# Autodesk Inventor assembly: P3_device(Main)
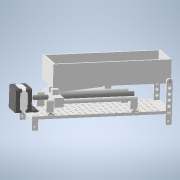
[picture p0: Inventor's stored thumbnail of the model, 180x180]
Saved by Autodesk Inventor 2021 (Build 250183000, 183)
## iProperties
Created: 2021-02-05
Part Number: P3_device(Main)
Document SubType Name: Assembly
Designer: chris
Author: chris
## Documents named in this file (13)
- C:\Users\chris\Desktop\Mon-38_P3_CAD_Files\Project 3 Device\P3_device(Main).iam
- C:\Users\chris\Desktop\Mon-38_P3_CAD_Files\Project 3 Device\Q-Bot baseplate\Mounting Platform.iam
- C:\Users\chris\Desktop\Mon-38_P3_CAD_Files\Project 3 Device\Rotary Actuator\Stepper Motor.iam
- C:\Users\chris\Desktop\Mon-38_P3_CAD_Files\Project 3 Device\Screws\Short Screw (Stepper Motor & Linear Actuator).ipt
- C:\Users\chris\Desktop\Mon-38_P3_CAD_Files\Project 3 Device\Main Screw.ipt
- C:\Users\chris\Desktop\Mon-38_P3_CAD_Files\Project 3 Device\moving_block_with_connector.iam
- C:\Users\chris\Desktop\Mon-38_P3_CAD_Files\Project 3 Device\Q-Bot baseplate\Additional\Mounting Platform Axle.ipt
- C:\Users\chris\Desktop\Mon-38_P3_CAD_Files\Project 3 Device\hopper_with_connector.iam
- C:\Users\chris\Desktop\Mon-38_P3_CAD_Files\Project 3 Device\rod.ipt
- C:\Users\chris\Desktop\Mon-38_P3_CAD_Files\Project 3 Device\rod_axle.ipt
- C:\Users\chris\Desktop\Mon-38_P3_CAD_Files\Project 3 Device\Containers\Metal_Container.ipt
- C:\Users\chris\Desktop\Mon-38_P3_CAD_Files\Project 3 Device\Supporting-Rod.ipt
- C:\Users\chris\Desktop\Mon-38_P3_CAD_Files\Project 3 Device\Supporting-Rod(mirror).ipt
## Components (21 placed, 12 different names)
1. Mounting Platform:1 [sub-assembly] — Mate:1, Mate:2, Mate:3, Mate:13, Mate:14, Angle:1, Mate:27, Mate:28, Mate:29, Mate:31, Mate:32, Mate:33
2. Stepper Motor:1 [sub-assembly] — Mate:1, Mate:2, Mate:3, Insert:1, Insert:2, Insert:3, Mate:4, Mate:5, Mate:6
3. Short Screw (Stepper Motor & Linear Actuator):1 — Insert:1
4. Short Screw (Stepper Motor & Linear Actuator):2 — Insert:2
5. Short Screw (Stepper Motor & Linear Actuator):3 — Insert:3
6. Main Screw:1 — Mate:4, Mate:5, Mate:6, Mate:7, Rotation/Translation:1
7. moving_block_with_connector:1 [sub-assembly] — Mate:7, Rotation/Translation:1, Mate:21, Mate:23, Mate:25, Flush:1, Mate:30, Mate:34, Mate:35
8. Short Screw (Stepper Motor & Linear Actuator):4 — Insert:9
9. Short Screw (Stepper Motor & Linear Actuator):5 — Insert:8
10. Mounting Platform Axle:1 — Mate:13, Mate:14, Mate:20
11. Short Screw (Stepper Motor & Linear Actuator):6 — Insert:11
12. Short Screw (Stepper Motor & Linear Actuator):7 — Insert:10
13. hopper_with_connector:1 [sub-assembly] — Mate:20, Mate:22, Mate:24, Mate:26, Flush:2, Angle:1
14. rod:1 — Mate:21, Mate:22, Mate:23, Mate:24
15. rod_axle:1 — Mate:26, Flush:2
16. rod_axle:2 — Mate:25, Flush:1
17. Metal_Container:1
18. Metal_Container:2
19. Metal_Container:3
20. Supporting-Rod:1 — Mate:27, Mate:28, Mate:29, Insert:8, Insert:9, Mate:30, Mate:35
21. Supporting-Rod(mirror):1 — Mate:31, Mate:32, Mate:33, Insert:10, Insert:11, Mate:34
## Relationships (36: Mate 25, Insert 7, Flush 2, RelateRotateTranslate 1, Angle 1)
- Mate:1: Mounting Platform:1 ↔ Stepper Motor:1
- Mate:2: Mounting Platform:1 ↔ Stepper Motor:1
- Mate:3: Mounting Platform:1 ↔ Stepper Motor:1
- Insert:1: Stepper Motor:1 ↔ Short Screw (Stepper Motor & Linear Actuator):1
- Insert:2: Stepper Motor:1 ↔ Short Screw (Stepper Motor & Linear Actuator):2
- Insert:3: Stepper Motor:1 ↔ Short Screw (Stepper Motor & Linear Actuator):3
- Mate:4: Stepper Motor:1 ↔ Main Screw:1
- Mate:5: Stepper Motor:1 ↔ Main Screw:1
- Mate:6: Stepper Motor:1 ↔ Main Screw:1
- Mate:7: Main Screw:1 ↔ moving_block_with_connector:1
- Mate:13: Mounting Platform:1 ↔ Mounting Platform Axle:1
- Mate:14 (1.2 mm): Mounting Platform:1 ↔ Mounting Platform Axle:1
- Rotation/Translation:1 [RelateRotateTranslate] (31.416 mm): Main Screw:1 ↔ moving_block_with_connector:1
- Mate:20: Mounting Platform Axle:1 ↔ hopper_with_connector:1
- Mate:21: moving_block_with_connector:1 ↔ rod:1
- Mate:22: hopper_with_connector:1 ↔ rod:1
- Mate:23 (1 mm): moving_block_with_connector:1 ↔ rod:1
- Mate:24 (1 mm): hopper_with_connector:1 ↔ rod:1
- Mate:25: moving_block_with_connector:1 ↔ rod_axle:2
- Flush:1 (-1 mm): moving_block_with_connector:1 ↔ rod_axle:2
- Mate:26: hopper_with_connector:1 ↔ rod_axle:1
- Flush:2 (-1 mm): hopper_with_connector:1 ↔ rod_axle:1
- Angle:1 (0 deg): Mounting Platform:1 ↔ hopper_with_connector:1
- Mate:27: Mounting Platform:1 ↔ Supporting-Rod:1
- Mate:28: Mounting Platform:1 ↔ Supporting-Rod:1
- Mate:29: Mounting Platform:1 ↔ Supporting-Rod:1
- Insert:8: Short Screw (Stepper Motor & Linear Actuator):5 ↔ Supporting-Rod:1
- Insert:9: Short Screw (Stepper Motor & Linear Actuator):4 ↔ Supporting-Rod:1
- Mate:30 (19.275 mm): moving_block_with_connector:1 ↔ Supporting-Rod:1
- Mate:31: Mounting Platform:1 ↔ Supporting-Rod(mirror):1
- Mate:32: Mounting Platform:1 ↔ Supporting-Rod(mirror):1
- Mate:33: Mounting Platform:1 ↔ Supporting-Rod(mirror):1
- Insert:10: Short Screw (Stepper Motor & Linear Actuator):7 ↔ Supporting-Rod(mirror):1
- Insert:11: Short Screw (Stepper Motor & Linear Actuator):6 ↔ Supporting-Rod(mirror):1
- Mate:34: moving_block_with_connector:1 ↔ Supporting-Rod(mirror):1
- Mate:35: moving_block_with_connector:1 ↔ Supporting-Rod:1
